# Autodesk Inventor assembly: Omni-Wheel_r1
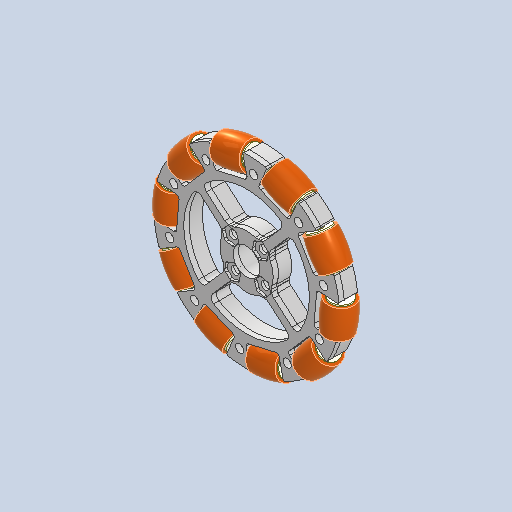
[picture p0: Inventor's stored thumbnail of the model, 512x512]
Saved by Autodesk Inventor 2025 (Build 290162000, 162)
## iProperties
Created: 2024-06-25
Part Number: Omni-Wheel_r1
Document SubType Name: Assembly
Designer: 8326d
Author: 8326d
## Documents named in this file (6)
- C:\Users\8326d\Documents\hobby\CAD\General-Purpose-Robot\Omni-Wheel\Omni-Wheel_r1.iam
- C:\Users\8326d\Documents\hobby\CAD\General-Purpose-Robot\Omni-Wheel\3D_taru-core.ipt
- C:\Users\8326d\Documents\hobby\CAD\General-Purpose-Robot\Omni-Wheel\pin.ipt
- C:\Users\8326d\Documents\hobby\CAD\General-Purpose-Robot\Omni-Wheel\pom_bush.ipt
- C:\Users\8326d\Documents\hobby\CAD\General-Purpose-Robot\Omni-Wheel\T5.0_base1.ipt
- C:\Users\8326d\Documents\hobby\CAD\General-Purpose-Robot\Omni-Wheel\T2.0_base2.ipt
## Components (42 placed, 5 different names)
1. T5.0_base1:1 — メイト:2, 正接:1, 正接:2, メイト:3, メイト:4, フラッシュ:1, 挿入:3, 挿入:4
2. T2.0_base2:1 — 挿入:3, 挿入:4
3. 3D_taru-core:1 — メイト:1, 挿入:1, 挿入:2
4. pom_bush:1 — 挿入:2
5. pin:1 — メイト:1, メイト:2, 正接:1, 正接:2
6. pom_bush:2 — 挿入:1, メイト:3
7. 3D_taru-core:2
8. pom_bush:4
9. pin:2
10. pom_bush:5
11. 3D_taru-core:3
12. pom_bush:6
13. pin:3
14. pom_bush:7
15. 3D_taru-core:4
16. pom_bush:8
17. pin:4
18. pom_bush:9
19. 3D_taru-core:5
20. pom_bush:10
21. pin:5
22. pom_bush:11
23. 3D_taru-core:6
24. pom_bush:12
25. pin:6
26. pom_bush:13
27. 3D_taru-core:7
28. pom_bush:14
29. pin:7
30. pom_bush:15
31. 3D_taru-core:8
32. pom_bush:16
33. pin:8
34. pom_bush:17
35. 3D_taru-core:9
36. pom_bush:18
37. pin:9
38. pom_bush:19
39. 3D_taru-core:10
40. pom_bush:20
41. pin:10
42. pom_bush:21
## Component patterns: (10 elements, first: 3D_taru-core:1 + pom_bush:1 + pin:1 + pom_bush:2)
## Relationships (11: Mate 4, Insert 4, Tangent 2, Flush 1)
- メイト:1 [Mate]: 3D_taru-core:1 ↔ pin:1
- メイト:2 [Mate]: T5.0_base1:1 ↔ pin:1
- 正接:1 [Tangent]: T5.0_base1:1 ↔ pin:1
- 正接:2 [Tangent]: T5.0_base1:1 ↔ pin:1
- 挿入:1 [Insert]: 3D_taru-core:1 ↔ pom_bush:2
- メイト:3 [Mate]: T5.0_base1:1 ↔ pom_bush:2
- 挿入:2 [Insert]: 3D_taru-core:1 ↔ pom_bush:1
- メイト:4 [Mate]: T5.0_base1:1
- フラッシュ:1 [Flush] (1.5 mm): T5.0_base1:1
- 挿入:3 [Insert]: T5.0_base1:1 ↔ T2.0_base2:1
- 挿入:4 [Insert]: T5.0_base1:1 ↔ T2.0_base2:1
